# Autodesk Inventor assembly: Lidarsee_v2
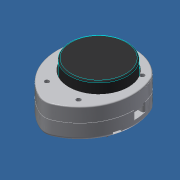
[picture p0: Inventor's stored thumbnail of the model, 180x180]
Saved by Autodesk Inventor 2016 (Build 200138000, 138)
## iProperties
Created: 2017-05-10
Part Number: Lidarsee_v2
Material: Generisch
Document SubType Name: Assembly
Designer: 4ndreas
Author: 4ndreas
## Documents named in this file (6)
- C:\Users\4ndreas\Documents\Inventor\lidarsee\Lidarsee_v2.iam
- C:\Users\4ndreas\Documents\Inventor\lidarsee\LidarseeCase_v2_A.ipt
- C:\Users\4ndreas\Documents\Inventor\lidarsee\Lidar_v2.ipt
- C:\Users\4ndreas\Documents\Inventor\lidarsee\LidarseeCase_v2_B.ipt
- C:\Users\4ndreas\Documents\Inventor\lidarsee\LidarseeCase_v2_C.ipt
- C:\Users\4ndreas\Documents\Inventor\lidarsee\Mount.ipt
## Components (6 placed, 5 different names)
1. LidarseeCase_v2_A:1 — Fluchtend:1, Fluchtend:2, Fluchtend:3, Passend:1, Passend:2, Passend:3, Passend:4, Passend:7, Passend:8, Passend:9, Passend:10
2. Lidar_v2:1 — Passend:1, Passend:2, Passend:3, Passend:5
3. LidarseeCase_v2_B:1 — Passend:4, Passend:5, Passend:10
4. LidarseeCase_v2_C:1 — Passend:7, Passend:8, Passend:9, Passend:11, Passend:12, Passend:13, Passend:14, Passend:15, Passend:16
5. Mount:1 — Passend:11, Passend:12, Passend:13
6. Mount:2 — Passend:14, Passend:15, Passend:16
## Relationships (18: Mate 15, Flush 3)
- Fluchtend:1 [Flush]: LidarseeCase_v2_A:1
- Fluchtend:2 [Flush]: LidarseeCase_v2_A:1
- Fluchtend:3 [Flush]: LidarseeCase_v2_A:1
- Passend:1 [Mate]: LidarseeCase_v2_A:1 ↔ Lidar_v2:1
- Passend:2 [Mate]: LidarseeCase_v2_A:1 ↔ Lidar_v2:1
- Passend:3 [Mate]: LidarseeCase_v2_A:1 ↔ Lidar_v2:1
- Passend:4 [Mate]: LidarseeCase_v2_A:1 ↔ LidarseeCase_v2_B:1
- Passend:5 [Mate]: Lidar_v2:1 ↔ LidarseeCase_v2_B:1
- Passend:7 [Mate]: LidarseeCase_v2_A:1 ↔ LidarseeCase_v2_C:1
- Passend:8 [Mate]: LidarseeCase_v2_A:1 ↔ LidarseeCase_v2_C:1
- Passend:9 [Mate]: LidarseeCase_v2_A:1 ↔ LidarseeCase_v2_C:1
- Passend:10 [Mate]: LidarseeCase_v2_A:1 ↔ LidarseeCase_v2_B:1
- Passend:11 [Mate]: LidarseeCase_v2_C:1 ↔ Mount:1
- Passend:12 [Mate]: LidarseeCase_v2_C:1 ↔ Mount:1
- Passend:13 [Mate]: LidarseeCase_v2_C:1 ↔ Mount:1
- Passend:14 [Mate]: LidarseeCase_v2_C:1 ↔ Mount:2
- Passend:15 [Mate]: LidarseeCase_v2_C:1 ↔ Mount:2
- Passend:16 [Mate]: LidarseeCase_v2_C:1 ↔ Mount:2
